# Autodesk Inventor assembly: DriverStation-ver2-1111-2021
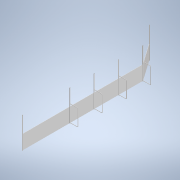
[picture p0: Inventor's stored thumbnail of the model, 180x180]
Saved by Autodesk Inventor 2021 (Build 250183000, 183)
## iProperties
Created: 2021-03-02
Part Number: DriverStation-ver2-1111-2021
Document SubType Name: Assembly
Designer: CMurray
Author: CMurray
## Documents named in this file (6)
- F:\PHRC CADD 2021\2021 Game Design Challenge\Player Station\Assemblies\DriverStation-ver2-1111-2021.iam
- F:\PHRC CADD 2021\2021 Game Design Challenge\Player Station\Parts\StationBase-ver1-1111-2021.ipt
- F:\PHRC CADD 2021\2021 Game Design Challenge\Player Station\Parts\StationDivider-ver1-1111-2021.iam
- F:\PHRC CADD 2021\2021 Game Design Challenge\Player Station\Parts\HPStationBase-ver1-1111-2021.ipt
- F:\PHRC CADD 2021\2021 Game Design Challenge\Player Station\Parts\StationDividerNoArm-ver1-1111-2021.iam
- F:\PHRC CADD 2021\2021 Game Design Challenge\Player Station\Parts\PSHalfWall-ver2-1111-2021.ipt
## Components (11 placed, 5 different names)
1. StationBase-ver1-1111-2021:1 — Mate:1, Flush:1, Flush:2, Flush:3, Mate:2, Flush:4, Flush:7, Flush:8, Flush:11, Flush:12
2. StationDivider-ver1-1111-2021:1 [sub-assembly] — Mate:1, Flush:1, Flush:2, Mate:6
3. StationDivider-ver1-1111-2021:2 [sub-assembly] — Flush:3, Mate:2, Flush:4, Mate:4, Angle:2
4. StationBase-ver1-1111-2021:2 — Mate:4, Flush:7, Flush:8, Mate:9, Flush:16, Flush:17, Angle:3
5. StationBase-ver1-1111-2021:3 — Flush:11, Flush:12, Mate:6, Flush:19, Flush:20
6. StationDivider-ver1-1111-2021:4 [sub-assembly] — Mate:12
7. StationDivider-ver1-1111-2021:6 [sub-assembly] — Mate:9, Flush:16, Angle:2, Mate:10, Angle:4
8. HPStationBase-ver1-1111-2021:1 — Mate:10, Flush:17, Angle:3, Mate:11, Flush:18
9. StationDividerNoArm-ver1-1111-2021:1 [sub-assembly] — Mate:11, Angle:4, Flush:18
10. PSHalfWall-ver2-1111-2021:1 — Flush:19, Flush:20, Mate:12, Mate:13, Flush:21, Flush:22
11. StationDividerNoArm-ver1-1111-2021:2 [sub-assembly] — Mate:13, Flush:21, Flush:22
## Relationships (30: Flush 17, Mate 10, Angle 3)
- Mate:1: StationBase-ver1-1111-2021:1 ↔ StationDivider-ver1-1111-2021:1
- Flush:1: StationBase-ver1-1111-2021:1 ↔ StationDivider-ver1-1111-2021:1
- Flush:2: StationBase-ver1-1111-2021:1 ↔ StationDivider-ver1-1111-2021:1
- Flush:3: StationBase-ver1-1111-2021:1 ↔ StationDivider-ver1-1111-2021:2
- Mate:2: StationBase-ver1-1111-2021:1 ↔ StationDivider-ver1-1111-2021:2
- Flush:4: StationBase-ver1-1111-2021:1 ↔ StationDivider-ver1-1111-2021:2
- Mate:4: StationDivider-ver1-1111-2021:2 ↔ StationBase-ver1-1111-2021:2
- Flush:7: StationBase-ver1-1111-2021:1 ↔ StationBase-ver1-1111-2021:2
- Flush:8: StationBase-ver1-1111-2021:1 ↔ StationBase-ver1-1111-2021:2
- [Mate]: StationBase-ver1-1111-2021:3 ↔ StationDivider-ver1-1111-2021:4
- [Flush]: StationBase-ver1-1111-2021:3 ↔ StationDivider-ver1-1111-2021:4
- [Flush]: StationBase-ver1-1111-2021:3 ↔ StationDivider-ver1-1111-2021:4
- Flush:11: StationBase-ver1-1111-2021:1 ↔ StationBase-ver1-1111-2021:3
- Flush:12: StationBase-ver1-1111-2021:1 ↔ StationBase-ver1-1111-2021:3
- Mate:6: StationDivider-ver1-1111-2021:1 ↔ StationBase-ver1-1111-2021:3
- Mate:9: StationBase-ver1-1111-2021:2 ↔ StationDivider-ver1-1111-2021:6
- Flush:16: StationBase-ver1-1111-2021:2 ↔ StationDivider-ver1-1111-2021:6
- Angle:2 (0 deg): StationDivider-ver1-1111-2021:2 ↔ StationDivider-ver1-1111-2021:6
- Mate:10: StationDivider-ver1-1111-2021:6 ↔ HPStationBase-ver1-1111-2021:1
- Flush:17: StationBase-ver1-1111-2021:2 ↔ HPStationBase-ver1-1111-2021:1
- Angle:3 (35 deg): StationBase-ver1-1111-2021:2 ↔ HPStationBase-ver1-1111-2021:1
- Mate:11: HPStationBase-ver1-1111-2021:1 ↔ StationDividerNoArm-ver1-1111-2021:1
- Angle:4 (0 deg): StationDivider-ver1-1111-2021:6 ↔ StationDividerNoArm-ver1-1111-2021:1
- Flush:18: HPStationBase-ver1-1111-2021:1 ↔ StationDividerNoArm-ver1-1111-2021:1
- Flush:19: StationBase-ver1-1111-2021:3 ↔ PSHalfWall-ver2-1111-2021:1
- Flush:20: StationBase-ver1-1111-2021:3 ↔ PSHalfWall-ver2-1111-2021:1
- Mate:12: StationDivider-ver1-1111-2021:4 ↔ PSHalfWall-ver2-1111-2021:1
- Mate:13: PSHalfWall-ver2-1111-2021:1 ↔ StationDividerNoArm-ver1-1111-2021:2
- Flush:21: PSHalfWall-ver2-1111-2021:1 ↔ StationDividerNoArm-ver1-1111-2021:2
- Flush:22: PSHalfWall-ver2-1111-2021:1 ↔ StationDividerNoArm-ver1-1111-2021:2
## Named parameters: d12_d0 = 0 mm, d13_d1 = 0 mm, d14_d2 = 0 mm
